# Autodesk Inventor assembly: CNC_01
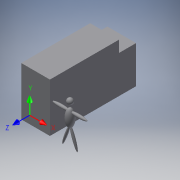
[picture p0: Inventor's stored thumbnail of the model, 180x180]
Saved by Autodesk Inventor 2019.4 (Build 234330000, 330)
## iProperties
Created: 2019-10-31
Part Number: CNC_01
Document SubType Name: Assembly
Designer: holecep
Mass: 1.00387e+07 g
Surface Area: 326861 cm^2
Volume: 1.00387e+07 cm^3
Density: 1 g/cm^3
description: 0:0:Test
manufacturer: 0:0:Holecep
model: 0:0:CNC
url: 0:0:https://github.com/slavikz-centrum/da-devcon2019
Author: holecep
## Documents named in this file (4)
- D:\Git\slavikz-centrum\da-devcon2019\inventorPlugins\InventorSatExport\DebugPluginLocally\inputFiles\CNC_01.iam
- C:\Users\holecep\Documents\Inventor\RFA\Demo1\CNC.ipt
- C:\Users\holecep\Documents\Inventor\RFA\Demo1\human.ipt
- C:\Users\holecep\Documents\Inventor\RFA\Demo1\CNC_01_Substitute_1.ipt
## Components (3 placed, 3 different names)
1. CNC:1 — Mate:1, Mate:2, Mate:3
2. human:1 — Mate:1, Mate:2, Mate:3
3. CNC_01_Substitute_1:1
## Relationships (3: Mate 3)
- Mate:1 (889 mm): CNC:1 ↔ human:1
- Mate:2: CNC:1 ↔ human:1
- Mate:3: CNC:1 ↔ human:1
## Named parameters: param1 = 889 mm
